# Autodesk Inventor assembly: IPT_TRACK_assembly
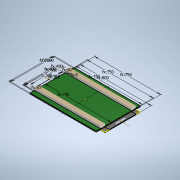
[picture p0: Inventor's stored thumbnail of the model, 180x180]
Saved by Autodesk Inventor 2021 (Build 250183000, 183)
## iProperties
Created: 2021-02-13
Part Number: IPT_TRACK_assembly
Document SubType Name: Assembly
Designer: phamv
Author: phamv
## Documents named in this file (5)
- C:\Users\phamv\OneDrive\UoA\2020 SUMMER\2020-srw-rc-car\CoilDesign\DEXTER_WORKSPACE\CAD stuff\Final_CAD\IPT_TRACK_assembly.iam
- C:\Users\phamv\OneDrive\UoA\2020 SUMMER\2020-srw-rc-car\CoilDesign\DEXTER_WORKSPACE\CAD stuff\Final_CAD\ferrite_layer_dex_1R1.ipt
- C:\Users\phamv\OneDrive\UoA\2020 SUMMER\2020-srw-rc-car\CoilDesign\DEXTER_WORKSPACE\CAD stuff\Final_CAD\coil_layer_1R1.ipt
- C:\Users\phamv\OneDrive\UoA\2020 SUMMER\2020-srw-rc-car\CoilDesign\DEXTER_WORKSPACE\CAD stuff\Final_CAD\track_surface_layer.ipt
- C:\Users\phamv\OneDrive\UoA\2020 SUMMER\2020-srw-rc-car\CoilDesign\DEXTER_WORKSPACE\CAD stuff\Final_CAD\track_walls.ipt
## Components (5 placed, 4 different names)
1. track_surface_layer:1 — Rigid:2, Rigid:3, Rigid:4
2. coil_layer_1R1:1 — Rigid:1, Rigid:2
3. ferrite_layer_dex_1R1:1 — Rigid:1
4. track_walls:1 — Rigid:3
5. track_walls:2 — Rigid:4
## Relationships (4: WeldJoint 4)
- Rigid:1 [WeldJoint]: coil_layer_1R1:1 ↔ ferrite_layer_dex_1R1:1
- Rigid:2 [WeldJoint]: track_surface_layer:1 ↔ coil_layer_1R1:1
- Rigid:3 [WeldJoint]: track_surface_layer:1 ↔ track_walls:1
- Rigid:4 [WeldJoint]: track_surface_layer:1 ↔ track_walls:2
## Named parameters: track_length = 800 mm, track_width = 300 mm, edge_gap_distance = 14.5 mm, ferrite_length = 109 mm, ferrite_width = 15 mm, parameter_5 = 126 mm, number_of_ferrites = 7, layer_width = 400 mm, bolt_diameter = 8 mm, layer_length = 800 mm, real_sheet_width = 500 mm, ferrite_height = 8 mm, parameter_2 = 30 mm, parameter_6 = 120 mm, number_of_bolts = 5, x_offset_for_bolts = 20 mm, y_offset_for_bolts = 175 mm, wire_diameter = 4.5 mm, distance_between_wires = 18.6 mm, distance_between_wires_edge = 8.25 mm, bend_radius_inner = 15 mm, bend_radius_outer = 18.5 mm, wall_length = 800 mm, wall_width = 50 mm, wall_thickness = 25 mm
